# Autodesk Inventor assembly: Chassis
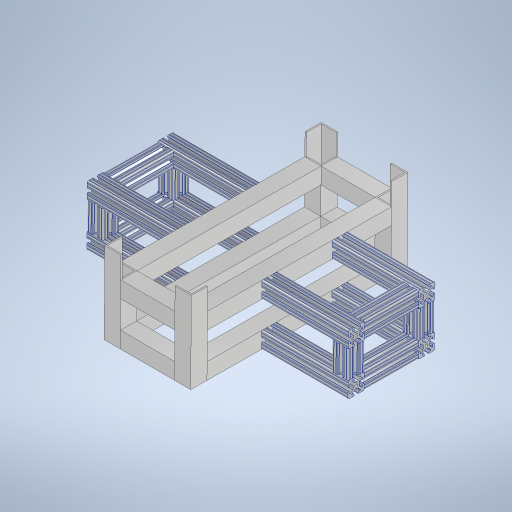
[picture p0: Inventor's stored thumbnail of the model, 512x512]
Saved by Autodesk Inventor 2023 (Build 270158000, 158)
## iProperties
Created: 2022-04-29
Part Number: Chassis
Document SubType Name: Assembly
Designer: Nebil Oumer
Mass: 8270.51 g
Surface Area: 16474 cm^2
Volume: 3063.15 cm^3
Density: 2.7 g/cm^3
Author: Nebil Oumer
## Documents named in this file (3)
- C:\Users\seene\Desktop\Stony Brook\SBRT\testRoboRescue\Chassis\Frame\Chassis.iam
- C:\Users\seene\Desktop\Stony Brook\SBRT\testRoboRescue\Chassis\Frame\testRoboRescue_Chassis_Frame.iam
- C:\Users\seene\Desktop\Stony Brook\SBRT\testRoboRescue\Chassis\Frame\8020ChassisSupport.iam
## Components (3 placed, 2 different names)
1. testRoboRescue_Chassis_Frame:1 [sub-assembly] — Mate:1, Flush:3, Flush:4, Mate:2
2. 8020ChassisSupport:1 [sub-assembly] — Flush:4, Mate:2
3. 8020ChassisSupport:2 [sub-assembly] — Mate:1, Flush:3
## Relationships (4: Mate 2, Flush 2)
- Mate:1: testRoboRescue_Chassis_Frame:1 ↔ 8020ChassisSupport:2
- Flush:3: testRoboRescue_Chassis_Frame:1 ↔ 8020ChassisSupport:2
- Flush:4: testRoboRescue_Chassis_Frame:1 ↔ 8020ChassisSupport:1
- Mate:2: testRoboRescue_Chassis_Frame:1 ↔ 8020ChassisSupport:1
